# Autodesk Inventor assembly: shaft holder
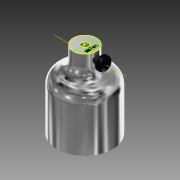
[picture p0: Inventor's stored thumbnail of the model, 180x180]
Saved by Autodesk Inventor 2013 (Build 170138000, 138)
## iProperties
Created: 2015-04-06
Part Number: shaft holder
Document SubType Name: Assembly
Designer: Nico
Author: Nico
## Documents named in this file (4)
- D:\Documents\Inventor\Fish Rod laquer Machine\shaft holder.iam
- D:\Documents\Inventor\Fish Rod laquer Machine\support shaft end.ipt
- D:\Documents\Inventor\Content Center Files\R2013\en-US\ANSI B18.6.7M(00)\ANSI B18.6.7M - M3x0.5 x 6(4).ipt
- D:\Documents\Inventor\Content Center Files\R2013\en-US\ISO 4035(1)\ISO 4035 - M3DIN EN.ipt
## Components (3 placed, 3 different names)
1. support shaft end:1 — Mate:1, Mate:2
2. Cross Recessed Pan Head Machine Screw - Type I - Metric M3x0.5 x 6:1 — Mate:4, Mate:6
3. DIN EN 24035 M3:1 — Mate:2, Mate:3
## Relationships (6: Mate 6)
- Mate:1: support shaft end:1
- Mate:2: support shaft end:1 ↔ DIN EN 24035 M3:1
- Mate:3: DIN EN 24035 M3:1
- Mate:4: Cross Recessed Pan Head Machine Screw - Type I - Metric M3x0.5 x 6:1
- Mate:5
- Mate:6: Cross Recessed Pan Head Machine Screw - Type I - Metric M3x0.5 x 6:1
